# Autodesk Inventor assembly: X02598_LEGOmini_UpperBody
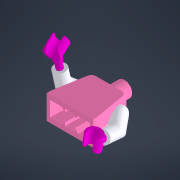
[picture p0: Inventor's stored thumbnail of the model, 180x180]
Saved by Autodesk Inventor 2022 (Build 260153000, 153)
## iProperties
Created: 2022-02-05
Part Number: X02598_LEGOmini_UpperBody
Document SubType Name: Assembly
Designer: Jason
Author: Jason
## Documents named in this file (5)
- C:\Users\User\Desktop\教材_LEGOmini_2022_20220218\X02598_LEGOmini_UpperBody.iam
- C:\Users\User\Desktop\教材_LEGOmini_2022_20220218\X02598_LEGOmini_UpperBody.ipt
- C:\Users\User\Desktop\教材_LEGOmini_2022_20220218\X02598_LEGOmini_BackArmL_G.ipt
- C:\Users\User\Desktop\教材_LEGOmini_2022_20220218\X02598_LEGOmini_BackArmR_G.ipt
- C:\Users\User\Desktop\教材_LEGOmini_2022_20220218\X02598_LEGOmini_FrontArm_Y.ipt
## Components (5 placed, 4 different names)
1. X02598_LEGOmini_UpperBody:1 — 插入:1, 插入:2
2. X02598_LEGOmini_BackArmL_G:1 — 插入:1, 貼合:2
3. X02598_LEGOmini_BackArmR_G:1 — 插入:2, 貼合:1
4. X02598_LEGOmini_FrontArm_Y:1 — 貼合:1
5. X02598_LEGOmini_FrontArm_Y:2 — 貼合:2
## Relationships (4: Insert 2, Mate 2)
- 插入:1 [Insert]: X02598_LEGOmini_UpperBody:1 ↔ X02598_LEGOmini_BackArmL_G:1
- 插入:2 [Insert]: X02598_LEGOmini_UpperBody:1 ↔ X02598_LEGOmini_BackArmR_G:1
- 貼合:1 [Mate]: X02598_LEGOmini_BackArmR_G:1 ↔ X02598_LEGOmini_FrontArm_Y:1
- 貼合:2 [Mate]: X02598_LEGOmini_BackArmL_G:1 ↔ X02598_LEGOmini_FrontArm_Y:2
